# Autodesk Inventor assembly: FE-00005
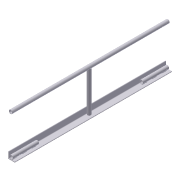
[picture p0: Inventor's stored thumbnail of the model, 180x180]
Saved by Autodesk Inventor 2012 (Build 160160000, 160)
## iProperties
Company: FIRST
Created: 2008-05-25
Part Number: FE-00005
Document SubType Name: Weldment
Designer: dfoster
Description: Field Rail
Weld Material: Welded Aluminum-6061
Title: Field Rail
Author: dfoster
## Documents named in this file (5)
- C:\Data Folder\FRC 2012 Field\Components\FE-00005.iam
- C:\Data Folder\FRC 2012 Field\Components\FE-00005-01.ipt
- C:\Data Folder\FRC 2012 Field\Components\FE-00005-02.ipt
- C:\Data Folder\FRC 2012 Field\Components\FE-00005-03.ipt
- C:\Data Folder\FRC 2012 Field\Components\FE-00005-04.ipt
## Components (5 placed, 4 different names)
1. FE-00005-01:1 — Tangent:1, Tangent:2, Flush:1, Tangent:3, Tangent:4, Flush:3, Mate:2, Angle:3, Tangent:5, Mate:3, Angle:4, Flush:5, Angle:6, Angle:8, Tangent:9
2. FE-00005-02:1 — Tangent:3, Tangent:4, Flush:3, Angle:8
3. FE-00005-02:2 — Tangent:1, Tangent:2, Flush:1, Angle:6
4. FE-00005-03:1 — Mate:2, Angle:3, Tangent:5, Mate:3
5. FE-00005-04:1 — Angle:4, Flush:5, Tangent:9
## Relationships (16: Tangent 7, Angle 4, Flush 3, Mate 2)
- Tangent:1: FE-00005-01:1 ↔ FE-00005-02:2
- Tangent:2: FE-00005-01:1 ↔ FE-00005-02:2
- Flush:1 (6.35 mm): FE-00005-01:1 ↔ FE-00005-02:2
- Tangent:3: FE-00005-01:1 ↔ FE-00005-02:1
- Tangent:4: FE-00005-01:1 ↔ FE-00005-02:1
- Flush:3 (6.35 mm): FE-00005-01:1 ↔ FE-00005-02:1
- Mate:2: FE-00005-01:1 ↔ FE-00005-03:1
- Angle:3 (180 deg): FE-00005-01:1 ↔ FE-00005-03:1
- Tangent:5: FE-00005-01:1 ↔ FE-00005-03:1
- Mate:3 (-914.4 mm): FE-00005-01:1 ↔ FE-00005-03:1
- [Tangent]: FE-00005-03:1 ↔ FE-00005-04:1
- Angle:4 (90 deg): FE-00005-01:1 ↔ FE-00005-04:1
- Flush:5: FE-00005-01:1 ↔ FE-00005-04:1
- Angle:6 (90 deg): FE-00005-01:1 ↔ FE-00005-02:2
- Angle:8 (-90 deg): FE-00005-01:1 ↔ FE-00005-02:1
- Tangent:9: FE-00005-01:1 ↔ FE-00005-04:1
